# Autodesk Inventor assembly: ведро крутое
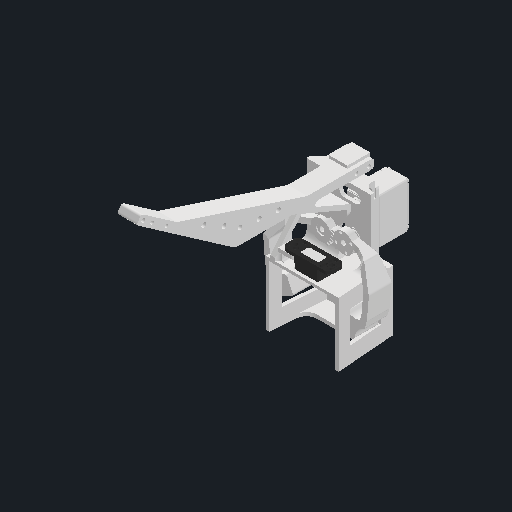
[picture p0: Inventor's stored thumbnail of the model, 512x512]
Saved by Autodesk Inventor 2025 (Build 290162000, 162)
## iProperties
Created: 2025-01-18
Part Number: ведро крутое
Document SubType Name: Assembly
Designer: Phantom
Author: Phantom
## Documents named in this file (7)
- C:\Users\Phantom\Desktop\Phantom16950\ведро крутое.iam
- C:\Users\Phantom\Desktop\Phantom16950\манипулятор 2.ipt
- C:\Users\Phantom\Desktop\Phantom16950\ведро.ipt
- C:\Users\Phantom\Desktop\Phantom16950\манипулятор 1.ipt
- C:\Users\Phantom\Desktop\Phantom16950\2000-0025-0002\2000-0025-0002.ipt
- C:\Users\Phantom\Downloads\Telegram Desktop\REV-31-1557\REV-31-1557.ipt
- C:\Users\Phantom\Desktop\Phantom16950\палка.ipt
## Components (6 placed, 6 different names)
1. манипулятор 2:1 — Совмещение:3, Совмещение:4
2. ведро:1 — Совмещение:2, Заподлицо:1, Совмещение:4, Совмещение:9, Совмещение:10, Совмещение:11, Заподлицо:2, Совмещение:12, Совмещение:13, Совмещение:14
3. манипулятор 1:1 — Совмещение:13, Совмещение:14
4. 2000-0025-0002:1 — Совмещение:2, Заподлицо:1, Совмещение:3
5. REV-31-1557:1 — Совмещение:9, Совмещение:10
6. палка:1 — Совмещение:11, Заподлицо:2, Совмещение:12
## Relationships (11: Mate 9, Flush 2)
- Совмещение:2 [Mate]: ведро:1 ↔ 2000-0025-0002:1
- Заподлицо:1 [Flush] (-1 mm): ведро:1 ↔ 2000-0025-0002:1
- Совмещение:3 [Mate]: манипулятор 2:1 ↔ 2000-0025-0002:1
- Совмещение:4 [Mate]: манипулятор 2:1 ↔ ведро:1
- Совмещение:9 [Mate]: ведро:1 ↔ REV-31-1557:1
- Совмещение:10 [Mate]: ведро:1 ↔ REV-31-1557:1
- Совмещение:11 [Mate]: ведро:1 ↔ палка:1
- Заподлицо:2 [Flush]: ведро:1 ↔ палка:1
- Совмещение:12 [Mate]: ведро:1 ↔ палка:1
- Совмещение:13 [Mate]: ведро:1 ↔ манипулятор 1:1
- Совмещение:14 [Mate]: ведро:1 ↔ манипулятор 1:1
